# Autodesk Inventor assembly: Assembly Line follower
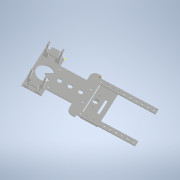
[picture p0: Inventor's stored thumbnail of the model, 180x180]
Saved by Autodesk Inventor 2022 (Build 260153000, 153)
## iProperties
Created: 2022-12-08
Part Number: Assembly Line follower
Document SubType Name: Assembly
Designer: Kilian De Ruyck
Author: Kilian De Ruyck
## Documents named in this file (5)
- C:\Users\Kilian De Ruyck\Documents\School 3de jaar\Semester 1\Syntheseproject\Assembly\Assembly Line follower.iam
- C:\Users\Kilian De Ruyck\Documents\School 3de jaar\Semester 1\Syntheseproject\FrameVer3\FrameVer5.ipt
- C:\Users\Kilian De Ruyck\Documents\School 3de jaar\Semester 1\Syntheseproject\FrameVer3\Sensoren plaat2.ipt
- C:\Users\Kilian De Ruyck\Documents\School 3de jaar\Semester 1\Syntheseproject\FrameVer3\Ball houder.ipt
- C:\Users\Kilian De Ruyck\Documents\School 3de jaar\Semester 1\Syntheseproject\Bracket onder\Bracket onder.ipt
## Components (5 placed, 4 different names)
1. FrameVer5:1 — Mate:1, Mate:2, Mate:3, Mate:7, Mate:8, Mate:9, Mate:10, Mate:11, Mate:12
2. Sensoren plaat2:1 — Mate:1, Mate:2, Mate:3, Mate:4, Mate:5, Mate:6
3. Ball houder:2 — Mate:4, Mate:5, Mate:6
4. Bracket onder:1 — Mate:8, Mate:9, Mate:10
5. Bracket onder:2 — Mate:7, Mate:11, Mate:12
## Relationships (12: Mate 12)
- Mate:1: FrameVer5:1 ↔ Sensoren plaat2:1
- Mate:2: FrameVer5:1 ↔ Sensoren plaat2:1
- Mate:3: FrameVer5:1 ↔ Sensoren plaat2:1
- Mate:4: Sensoren plaat2:1 ↔ Ball houder:2
- Mate:5: Sensoren plaat2:1 ↔ Ball houder:2
- Mate:6: Sensoren plaat2:1 ↔ Ball houder:2
- Mate:7: FrameVer5:1 ↔ Bracket onder:2
- Mate:8: FrameVer5:1 ↔ Bracket onder:1
- Mate:9: FrameVer5:1 ↔ Bracket onder:1
- Mate:10: FrameVer5:1 ↔ Bracket onder:1
- Mate:11: FrameVer5:1 ↔ Bracket onder:2
- Mate:12: FrameVer5:1 ↔ Bracket onder:2
